# Autodesk Inventor assembly: Robot
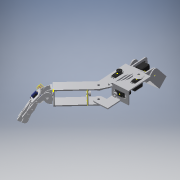
[picture p0: Inventor's stored thumbnail of the model, 180x180]
Saved by Autodesk Inventor 2018 (Build 220112000, 112)
## iProperties
Created: 2018-02-08
Part Number: Robot
Material: Générique
Document SubType Name: Assembly
Designer: Thomas
Author: Thomas
## Documents named in this file (6)
- D:\Users\Thomas\Desktop\Projet robot augmenté\robotConcept\Robot\Robot.iam
- D:\Users\Thomas\Desktop\Projet robot augmenté\robotConcept\Right forearm\RForearm+rotation.iam
- D:\Users\Thomas\Desktop\Projet robot augmenté\robotConcept\Right biceps\Rbiceps+servos.iam
- D:\Users\Thomas\Desktop\Projet robot augmenté\robotConcept\Shoulder\Shoulder1+servo.iam
- D:\Users\Thomas\Desktop\Projet robot augmenté\robotConcept\Shoulder\ShoulderPart2.ipt
- D:\Users\Thomas\Desktop\Projet robot augmenté\robotConcept\Hand\Full hand.iam
## Components (5 placed, 5 different names)
1. RForearm+rotation:1 [sub-assembly] — Rotation:1, Rotation:4
2. Rbiceps+servos:1 [sub-assembly] — Rotation:1, Placage:1, Rotation:2
3. Shoulder1+servo:1 [sub-assembly] — Placage:1, Rotation:2, Placage:2, Rotation:3
4. ShoulderPart2:1 — Placage:2, Rotation:3
5. Full hand:1 [sub-assembly] — Rotation:4
## Relationships (6: RevoluteJoint 4, Mate 2)
- Rotation:1 [RevoluteJoint]: RForearm+rotation:1 ↔ Rbiceps+servos:1
- Placage:1 [Mate]: Rbiceps+servos:1 ↔ Shoulder1+servo:1
- Rotation:2 [RevoluteJoint]: Rbiceps+servos:1 ↔ Shoulder1+servo:1
- Placage:2 [Mate]: Shoulder1+servo:1 ↔ ShoulderPart2:1
- Rotation:3 [RevoluteJoint]: Shoulder1+servo:1 ↔ ShoulderPart2:1
- Rotation:4 [RevoluteJoint]: RForearm+rotation:1 ↔ Full hand:1
